# Autodesk Inventor assembly: landing_gear
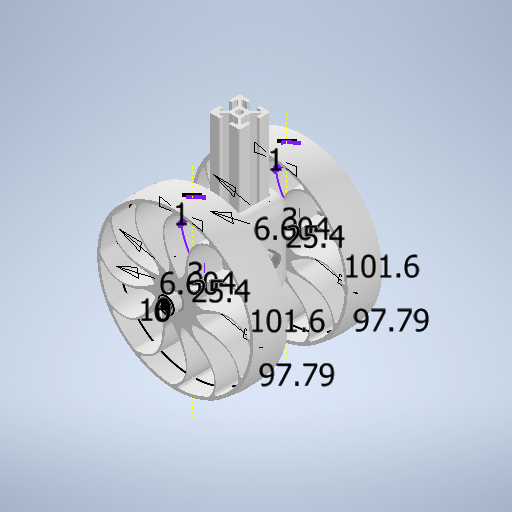
[picture p0: Inventor's stored thumbnail of the model, 512x512]
Saved by Autodesk Inventor 2025 (Build 290162000, 162)
## iProperties
Created: 2026-06-22
Part Number: landing_gear
Document SubType Name: Assembly
Designer: localadmin
Author: localadmin
## Documents named in this file (9)
- C:\Users\localadmin\github\SWIFT-UAV\System_development\Pelican\structural_model\v0.3.0\Parts\LandingGear\landing_gear.iam
- C:\Users\localadmin\Downloads\SWIFT-UAV-main\SWIFT-UAV-main\20x20alumnium.ipt
- C:\Users\localadmin\github\SWIFT-UAV\System_development\Pelican\structural_model\v0.3.0\Parts\LandingGear\arm_collar.ipt
- C:\Users\localadmin\github\SWIFT-UAV\System_development\Pelican\structural_model\v0.3.0\Parts\LandingGear\12spoke_wheel.ipt
- C:\Users\localadmin\Documents\Inventor\Content Center Files\R2025\en-US\ISO 7089\ISO 7089 - 6 - 140 HV(1).ipt
- C:\Users\localadmin\github\SWIFT-UAV\System_development\Pelican\structural_model\v0.3.0\Parts\LandingGear\m5_t_nut.ipt
- C:\Users\localadmin\Documents\Inventor\Content Center Files\R2025\en-US\ISO 4762(2)\ISO 4762 - M5 x 12ISO.ipt
- C:\Users\localadmin\github\SWIFT-UAV\System_development\Pelican\structural_model\v0.3.0\Parts\LandingGear\m6_bolt100mm.ipt
- C:\Users\localadmin\Documents\Inventor\Content Center Files\R2025\en-US\ISO 4032(2)\ISO 4032 - M6 - ISO.ipt
## Components (16 placed, 8 different names)
1. 20x20alumnium:1 — Mate:1, Mate:2, Mate:3, Mate:4, Mate:5, Mate:7, Mate:13
2. arm_collar:1 — Mate:2, Mate:3, Mate:4, Insert:1, Mate:9, Mate:12, Insert:5, Insert:6, Insert:7
3. 12spoke_wheel:1 — Insert:8, Mate:14, Insert:10
4. 12spoke_wheel:2 — Insert:3, Insert:9
5. ISO 7089 6:1 — Insert:7, Mate:14
6. ISO 7089 6:2 — Insert:10, Insert:11
7. ISO 7089 6:3 — Insert:1, Insert:4
8. ISO 7089 6:4 — Insert:3, Insert:4
9. ISO 7089 6:5 — Insert:8
10. ISO 7089 6:6 — Insert:9, Insert:12
11. m5_t_nut:1 — Mate:5, Mate:7, Mate:9
12. m5_t_nut:2 — Mate:12, Mate:13
13. ISO 4762 M5 x 12:1 — Insert:5
14. ISO 4762 M5 x 12:2 — Insert:6
15. m6_bolt100mm:1 — Insert:11
16. ISO 4032 M6:1 — Insert:12
## Relationships (21: Insert 11, Mate 10)
- Mate:1: 20x20alumnium:1
- Mate:2: 20x20alumnium:1 ↔ arm_collar:1
- Mate:3: 20x20alumnium:1 ↔ arm_collar:1
- Mate:4: 20x20alumnium:1 ↔ arm_collar:1
- Insert:1: arm_collar:1 ↔ ISO 7089 6:3
- Insert:3: 12spoke_wheel:2 ↔ ISO 7089 6:4
- Insert:4: ISO 7089 6:3 ↔ ISO 7089 6:4
- Mate:5: 20x20alumnium:1 ↔ m5_t_nut:1
- Mate:7: 20x20alumnium:1 ↔ m5_t_nut:1
- Mate:9: arm_collar:1 ↔ m5_t_nut:1
- Mate:12: arm_collar:1 ↔ m5_t_nut:2
- Mate:13: 20x20alumnium:1 ↔ m5_t_nut:2
- Insert:5: arm_collar:1 ↔ ISO 4762 M5 x 12:1
- Insert:6: arm_collar:1 ↔ ISO 4762 M5 x 12:2
- Insert:7: arm_collar:1 ↔ ISO 7089 6:1
- Insert:8: 12spoke_wheel:1 ↔ ISO 7089 6:5
- Insert:9: 12spoke_wheel:2 ↔ ISO 7089 6:6
- Mate:14: 12spoke_wheel:1 ↔ ISO 7089 6:1
- Insert:10: 12spoke_wheel:1 ↔ ISO 7089 6:2
- Insert:11: ISO 7089 6:2 ↔ m6_bolt100mm:1
- Insert:12: ISO 7089 6:6 ↔ ISO 4032 M6:1
